# Autodesk Inventor assembly: Right Hook Encoder Assembly
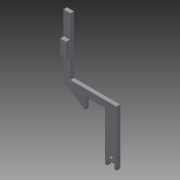
[picture p0: Inventor's stored thumbnail of the model, 180x180]
Saved by Autodesk Inventor 2013 (Build 170138000, 138)
## iProperties
Created: 2013-03-16
Part Number: Right Hook Encoder Assembly
Document SubType Name: Assembly
Designer: Arpan
Author: Arpan
## Documents named in this file (3)
- C:\Users\Arpan\Documents\GitHub\frc2013CAD\Midwest Climber\Right Hook Encoder Assembly.iam
- C:\Users\Arpan\Documents\GitHub\frc2013CAD\Midwest Climber\Right Climber Hook.ipt
- C:\Users\Arpan\Documents\GitHub\frc2013CAD\Midwest Climber\Limit Switch.ipt
## Components (2 placed, 2 different names)
1. Right Climber Hook:1 — Mate:1, Flush:1, Flush:2
2. Limit Switch:1 — Mate:1, Flush:1, Flush:2
## Relationships (3: Flush 2, Mate 1)
- Mate:1: Right Climber Hook:1 ↔ Limit Switch:1
- Flush:1 (1.5875 mm): Right Climber Hook:1 ↔ Limit Switch:1
- Flush:2 (63.5 mm): Right Climber Hook:1 ↔ Limit Switch:1
